# Autodesk Inventor assembly: Gesamtzusammensetzung
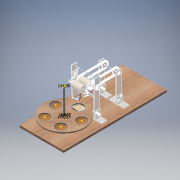
[picture p0: Inventor's stored thumbnail of the model, 180x180]
Saved by Autodesk Inventor 2018 (Build 220112000, 112)
## iProperties
Created: 2018-03-14
Part Number: Gesamtzusammensetzung
Material: Generisch
Document SubType Name: Assembly
Designer: Julian
Author: Julian
## Documents named in this file (8)
- C:\Users\Julian\Desktop\Schule\5AHME\Diplomarbeit\Git\fuettr_prototype\Mechanical\Inventorskizzen\Gesamtzusammensetzung.iam
- C:\Users\Julian\Desktop\Schule\5AHME\Diplomarbeit\Git\fuettr_prototype\Mechanical\Inventorskizzen\Grundplatte.ipt
- C:\Users\Julian\Desktop\Schule\5AHME\Diplomarbeit\Git\fuettr_prototype\Mechanical\Inventorskizzen\Plattenzusammensetzung.iam
- C:\Users\Julian\Desktop\Schule\5AHME\Diplomarbeit\Git\fuettr_prototype\Mechanical\Inventorskizzen\Förderband.iam
- C:\Users\Julian\Desktop\Schule\5AHME\Diplomarbeit\Git\fuettr_prototype\Mechanical\Inventorskizzen\Draht.ipt
- C:\Users\Julian\Desktop\Schule\5AHME\Diplomarbeit\Git\fuettr_prototype\Mechanical\Inventorskizzen\Draht_Halterung.ipt
- C:\Users\Julian\Documents\Inventor\Content Center Files\R2018\de-DE\CNS 4488\CNS 4488 - M3 x 8.ipt
- C:\Users\Julian\Documents\Inventor\Content Center Files\R2018\de-DE\GB_T 62.1-2004 A\GB_T 62.1 A - M3.ipt
## Components (10 placed, 7 different names)
1. Grundplatte:2 — Drehbar:1, Drehbar:2, Passend:1, Passend:3, Passend:4, Passend:5, Passend:7, Passend:8, Passend:10, Passend:11
2. Plattenzusammensetzung:1 [sub-assembly] — Drehbar:1
3. Förderband:1 [sub-assembly] — Drehbar:2, Drehbar:3, Drehbar:4, Drehbar:5, Drehbar:6
4. Draht:1 — Passend:1, Passend:2, Passend:6, Passend:9
5. Draht_Halterung:1 — Passend:2, Passend:3, Passend:4, Passend:5, Passend:6
6. Draht_Halterung:2 — Passend:7, Passend:8, Passend:9, Passend:10, Passend:11
7. CNS 4488 M3 x 8:1 — Drehbar:3
8. CNS 4488 M3 x 8:2 — Drehbar:4
9. Nut GB/T 62.1-2004 Type A A - M3:1 — Drehbar:6
10. Nut GB/T 62.1-2004 Type A A - M3:2 — Drehbar:5
## Relationships (17: Mate 11, RevoluteJoint 6)
- Drehbar:1 [RevoluteJoint]: Grundplatte:2 ↔ Plattenzusammensetzung:1
- Drehbar:2 [RevoluteJoint]: Grundplatte:2 ↔ Förderband:1
- Passend:1 [Mate]: Grundplatte:2 ↔ Draht:1
- Passend:2 [Mate]: Draht:1 ↔ Draht_Halterung:1
- Passend:3 [Mate]: Grundplatte:2 ↔ Draht_Halterung:1
- Passend:4 [Mate]: Grundplatte:2 ↔ Draht_Halterung:1
- Passend:5 [Mate]: Grundplatte:2 ↔ Draht_Halterung:1
- Passend:6 [Mate]: Draht:1 ↔ Draht_Halterung:1
- Passend:7 [Mate]: Grundplatte:2 ↔ Draht_Halterung:2
- Passend:8 [Mate]: Grundplatte:2 ↔ Draht_Halterung:2
- Passend:9 [Mate]: Draht:1 ↔ Draht_Halterung:2
- Passend:10 [Mate]: Grundplatte:2 ↔ Draht_Halterung:2
- Passend:11 [Mate]: Grundplatte:2 ↔ Draht_Halterung:2
- Drehbar:3 [RevoluteJoint]: Förderband:1 ↔ CNS 4488 M3 x 8:1
- Drehbar:4 [RevoluteJoint]: Förderband:1 ↔ CNS 4488 M3 x 8:2
- Drehbar:5 [RevoluteJoint]: Förderband:1 ↔ Nut GB/T 62.1-2004 Type A A - M3:2
- Drehbar:6 [RevoluteJoint]: Förderband:1 ↔ Nut GB/T 62.1-2004 Type A A - M3:1
